# Autodesk Inventor assembly: linear-guide-Hand
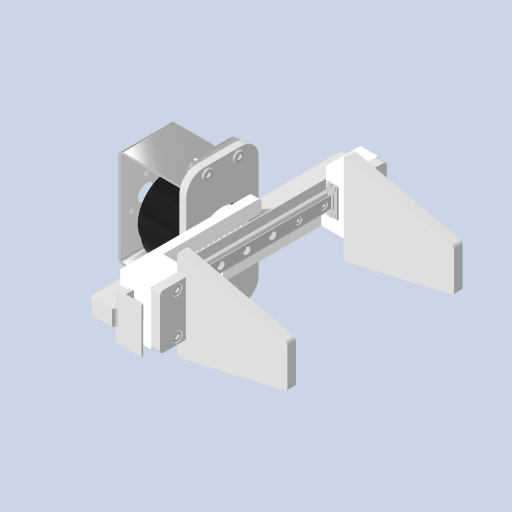
[picture p0: Inventor's stored thumbnail of the model, 512x512]
Saved by Autodesk Inventor 2023 (Build 270158000, 158)
## iProperties
Category: PARTsolutions
Company: MISUMI
Created: 2024-12-13
Part Number: linear-guide-Hand
Catalog Web Link: www.cadenas.de
Description: SSEBSLZ, SSEBSLZ-MX, SSE2BSLZ, SSE2BSLZ-MX-Miniature Linear Guides - Short Blocks - Light Preload/Slight Clearance - Standard Grade - Configurable
Vendor: MISUMI
Document SubType Name: Assembly
Designer: psAdmin
Manufacturer: MISUMI
Mass: 7.41683 g
Surface Area: 76.377 cm^2
Volume: 7.41683 cm^3
Density: 1 g/cm^3
PSOL_IDENT_0: {$CADENAS_DATA/23d-libs/misumi/metric/06_linear_guides/sebslz_asmtab.prj},252 {VTYP=3D},{STYP=ASSTAB
PSOL_IDENT_1: },{NB=SSE2BSLZ8-140},{LINA=SSE2BSLZ8-140},{NN=SSEBSLZ, SSEBSLZ-MX, SSE2BSLZ, SSE2BSLZ-MX},{DATE=04.0
PSOL_IDENT_2: 4.2024 07:13:14},{GEOMDATE=06.03.2024 06:19:47},{VERSION=},{LINEID=90},{WBVAR=TS,ST,MAT,MX,NOB,GREAS
PSOL_IDENT_3: E,L,ALT1,ALT4},{WBNUMERIC=L}  {NB=SSE2BSLZ8-140},{LINA=SSE2BSLZ8-140},{KT=DUMMY},{PN=SSE2BSLZ8-140},
PSOL_IDENT_4: {RT=B},{TS=Z},{TS1= 'Z','Standard' },{ST=S},{ST1='S', 'w/o Surface Treatment'},{TYPE=SSE2BSLZ},{MAT=
PSOL_IDENT_5: S},{MX=},{MXALG= '','w/o MX(Lubrication unit)' },{NOB=2},{H=8},{GREASE=},{GREASEALG='','Normal', 'L'
PSOL_IDENT_6: , 'L Type Greased ', 'G', 'G Type Greased', 'Y', 'Y Type Greased', 'H', 'H Type Greased'},{LT=Confi
PSOL_IDENT_7: gurable},{L=140},{HARD=56HRC~},{W=17},{L1=19.6},{B=12},{C=8},{SLL=M2x2.5},{L2=9.6},{K=6.5},{CBB=0.3}
PSOL_IDENT_8: ,{W1=7},{W2=5.0},{H1=4.7},{CAA=0.3},{DD1DD2HH=2.4x4.2x2.3},{F=15},{G=10},{ALT1=},{ALT1ALG= '', 'w/o
PSOL_IDENT_9: MC (Tapped Holes)' },{MC=M3},{MC1=3.0},{M=9},{LL=L},{L0=[56:69/1],[71:84/1],[86:99/1],[101:114/1],[1
PSOL_IDENT_10: 16:129/1],[131:144/1],[146:159/1],[161:174/1],[176:189/1],[191:204/1],[206:219/1],[221:234/1],[236:2
PSOL_IDENT_11: 49/1],[251:264/1],[266:279/1],[281:294/1],[296:309/1]},{REC1=   '','N/A'    },{ALT4=},{ALT4ALG= '','
PSOL_IDENT_12: N/A' },{PPATH=sebslz_series/sebslz_asmtpl.prj}
NB: SSE2BSLZ8-140
NN: SSEBSLZ, SSEBSLZ-MX, SSE2BSLZ, SSE2BSLZ-MX
NT: Miniature Linear Guides - Short Blocks - Light Preload/Slight Clearance - Standard Grade - Configurable
NBSYN: $PN.
LINA: SSE2BSLZ8-140
CATALOG: Misumi
PN: SSE2BSLZ8-140
MAT: Stainless Steel
MX: w/o MX(Lubrication unit)
NOB: 2
H: 8
GREASE: Normal
L: 140
W: 17
L1: 19.6
B: 12
C: 8
SLL: M2x2.5
L2: 9.6
K: 6.5
CBB: 0.3
W1: 7
W2: 5
H1: 4.7
CAA: 0.3
DD1DD2HH: 2.4x4.2x2.3
F: 15
G: 10
ALT1: w/o MC (Tapped Holes)
ALT4: N/A
SUPPLIER: MISUMI
ARTICLENO: SSE2BSLZ8-140
BOMINFO: SSE2BSLZ8-140
CREATOR: CADENAS GmbH
Title: SSE2BSLZ8-140
Author: Cadenas PARTsolutions
Comments: Miniature Linear Guides - Short Blocks - Light Preload/Slight Clearance - Standard Grade - Configurable
## Documents named in this file (16)
- D:\GitHub\inventor\syu-si\OfficeRobot\Hand\linear-guide-Hand.iam
- D:\GitHub\inventor\syu-si\OfficeRobot\ReadyMade\linear_guide\SSE2BSLZ8-140\SSE2BLZ8-140_r1.ipt
- D:\GitHub\inventor\syu-si\OfficeRobot\ReadyMade\linear_guide\SSE2BSLZ8-140\SEBSZ8_b.ipt
- D:\GitHub\inventor\syu-si\OfficeRobot\ReadyMade\linear_guide\SSE2BSLZ8-140\BOLT2-6.ipt
- D:\GitHub\inventor\syu-si\OfficeRobot\Hand\linear-gear.ipt
- D:\GitHub\inventor\syu-si\OfficeRobot\ReadyMade\Screw\CSH-316L-M2-6.ipt
- D:\GitHub\inventor\syu-si\OfficeRobot\Hand\fix-guide-motor.ipt
- D:\GitHub\inventor\syu-si\OfficeRobot\Hand\hand-gear.ipt
- D:\GitHub\inventor\syu-si\OfficeRobot\ReadyMade\Steadywin\GIM3505-8_with-driver.ipt
- D:\GitHub\inventor\syu-si\OfficeRobot\ReadyMade\Screw\CSH-316L-M2_5-6.ipt
- D:\GitHub\inventor\syu-si\OfficeRobot\Hand\sheet.ipt
- D:\GitHub\inventor\syu-si\OfficeRobot\Hand\hand_box2.ipt
- D:\GitHub\inventor\syu-si\OfficeRobot\Hand\nail.ipt
- D:\GitHub\inventor\syu-si\OfficeRobot\ReadyMade\Screw\FB-305530.ipt
- D:\GitHub\inventor\syu-si\OfficeRobot\ReadyMade\Screw\CBE3-5.ipt
- D:\GitHub\inventor\syu-si\OfficeRobot\ReadyMade\Screw\FB-2001.ipt
## Components (43 placed, 15 different names)
1. SSE2BLZ8-140_r1:1 — to_block_Z@1 <-> to_rail_Z@2, to_block_YZ@1 <-> to_rail_YZ@2, to_block_2_Z@1 <-> to_rail_Z@3, to_block_2_YZ@1 <-> to_rail_YZ@3, to_bolt_1_Z@1 <-> to_cp_Z@4, to_bolt_1_YZ@1 <-> to_cp_YZ@4, to_bolt_2_Z@1 <-> to_cp_Z@5, to_bolt_2_YZ@1 <-> to_cp_YZ@5, to_bolt_3_Z@1 <-> to_cp_Z@6, to_bolt_3_YZ@1 <-> to_cp_YZ@6, to_bolt_7_Z@1 <-> to_cp_Z@10, to_bolt_7_YZ@1 <-> to_cp_YZ@10, to_bolt_8_Z@1 <-> to_cp_Z@11, to_bolt_8_YZ@1 <-> to_cp_YZ@11, to_bolt_9_Z@1 <-> to_cp_Z@12, to_bolt_9_YZ@1 <-> to_cp_YZ@12, 挿入:6, 挿入:7, 挿入:13, 挿入:14, 挿入:15, 挿入:16, 挿入:17, 挿入:18, 挿入:19, 挿入:20
2. SEBSZ8_b:1 — to_block_Z@1 <-> to_rail_Z@2, to_block_YZ@1 <-> to_rail_YZ@2, メイト:15, メイト:16, メイト:17
3. SEBSZ8_b:2 — to_block_2_Z@1 <-> to_rail_Z@3, to_block_2_YZ@1 <-> to_rail_YZ@3, メイト:12, メイト:13, メイト:14
4. BOLT2-6:1 — to_bolt_1_Z@1 <-> to_cp_Z@4, to_bolt_1_YZ@1 <-> to_cp_YZ@4, 挿入:15
5. BOLT2-6:2 — to_bolt_2_Z@1 <-> to_cp_Z@5, to_bolt_2_YZ@1 <-> to_cp_YZ@5, 挿入:16
6. BOLT2-6:3 — to_bolt_3_Z@1 <-> to_cp_Z@6, to_bolt_3_YZ@1 <-> to_cp_YZ@6, 挿入:17
7. BOLT2-6:7 — to_bolt_7_Z@1 <-> to_cp_Z@10, to_bolt_7_YZ@1 <-> to_cp_YZ@10, 挿入:18
8. BOLT2-6:8 — to_bolt_8_Z@1 <-> to_cp_Z@11, to_bolt_8_YZ@1 <-> to_cp_YZ@11, 挿入:19
9. BOLT2-6:9 — to_bolt_9_Z@1 <-> to_cp_Z@12, to_bolt_9_YZ@1 <-> to_cp_YZ@12, 挿入:20
10. linear-gear:1 — メイト:12, メイト:13, メイト:14, 挿入:29, 挿入:30
11. linear-gear:2 — メイト:15, メイト:16, メイト:17, 挿入:27, 挿入:28
12. CSH-316L-M2-6:1
13. CSH-316L-M2-6:2
14. CSH-316L-M2-6:3
15. CSH-316L-M2-6:4
16. fix-guide-motor:1 — 挿入:6, 挿入:7, 挿入:8, 挿入:9, 挿入:10, 挿入:11, 挿入:12, 挿入:21, 挿入:22, 挿入:35, 挿入:36, 挿入:37, 挿入:38, 挿入:43, 挿入:44, 挿入:45, 挿入:46, 挿入:47, 挿入:48
17. 平歯車1:1 — 挿入:5
18. GIM3505-8_with-driver:1 — 挿入:5, 挿入:8, 挿入:9
19. CSH-316L-M2_5-6:1 — 挿入:10
20. CSH-316L-M2_5-6:2 — 挿入:12
21. CSH-316L-M2_5-6:3 — 挿入:11
22. sheet:1 — 挿入:13, 挿入:14
23. hand_box2:1 — 挿入:21, 挿入:22
24. nail:1 — 挿入:33, 挿入:34, 挿入:39, 挿入:40
25. nail:2 — 挿入:31, 挿入:32, 挿入:41, 挿入:42
26. FB-305530:2 — 挿入:30, 挿入:31
27. FB-305530:4 — 挿入:29, 挿入:32
28. FB-305530:5 — 挿入:28, 挿入:34
29. FB-305530:7 — 挿入:27, 挿入:33
30. CBE3-5:1 — 挿入:36
31. CBE3-5:2 — 挿入:35
32. CBE3-5:3 — 挿入:37
33. CBE3-5:4 — 挿入:38
34. CBE3-5:5 — 挿入:39
35. CBE3-5:6 — 挿入:40
36. CBE3-5:7 — 挿入:41
37. CBE3-5:8 — 挿入:42
38. FB-2001:1 — 挿入:48
39. FB-2001:2 — 挿入:47
40. FB-2001:3 — 挿入:46
41. FB-2001:4 — 挿入:45
42. FB-2001:5 — 挿入:44
43. FB-2001:6 — 挿入:43
## Relationships (66: Insert 44, Mate 14, Angle 8)
- to_block_Z@1 <-> to_rail_Z@2 [Mate]: SSE2BLZ8-140_r1:1 ↔ SEBSZ8_b:1
- to_block_YZ@1 <-> to_rail_YZ@2 [Angle] (180 deg): SSE2BLZ8-140_r1:1 ↔ SEBSZ8_b:1
- to_block_2_Z@1 <-> to_rail_Z@3 [Mate]: SSE2BLZ8-140_r1:1 ↔ SEBSZ8_b:2
- to_block_2_YZ@1 <-> to_rail_YZ@3 [Angle] (180 deg): SSE2BLZ8-140_r1:1 ↔ SEBSZ8_b:2
- to_bolt_1_Z@1 <-> to_cp_Z@4 [Mate]: SSE2BLZ8-140_r1:1 ↔ BOLT2-6:1
- to_bolt_1_YZ@1 <-> to_cp_YZ@4 [Angle] (0 deg): SSE2BLZ8-140_r1:1 ↔ BOLT2-6:1
- to_bolt_2_Z@1 <-> to_cp_Z@5 [Mate]: SSE2BLZ8-140_r1:1 ↔ BOLT2-6:2
- to_bolt_2_YZ@1 <-> to_cp_YZ@5 [Angle] (0 deg): SSE2BLZ8-140_r1:1 ↔ BOLT2-6:2
- to_bolt_3_Z@1 <-> to_cp_Z@6 [Mate]: SSE2BLZ8-140_r1:1 ↔ BOLT2-6:3
- to_bolt_3_YZ@1 <-> to_cp_YZ@6 [Angle] (0 deg): SSE2BLZ8-140_r1:1 ↔ BOLT2-6:3
- to_bolt_7_Z@1 <-> to_cp_Z@10 [Mate]: SSE2BLZ8-140_r1:1 ↔ BOLT2-6:7
- to_bolt_7_YZ@1 <-> to_cp_YZ@10 [Angle] (0 deg): SSE2BLZ8-140_r1:1 ↔ BOLT2-6:7
- to_bolt_8_Z@1 <-> to_cp_Z@11 [Mate]: SSE2BLZ8-140_r1:1 ↔ BOLT2-6:8
- to_bolt_8_YZ@1 <-> to_cp_YZ@11 [Angle] (0 deg): SSE2BLZ8-140_r1:1 ↔ BOLT2-6:8
- to_bolt_9_Z@1 <-> to_cp_Z@12 [Mate]: SSE2BLZ8-140_r1:1 ↔ BOLT2-6:9
- to_bolt_9_YZ@1 <-> to_cp_YZ@12 [Angle] (0 deg): SSE2BLZ8-140_r1:1 ↔ BOLT2-6:9
- メイト:12 [Mate]: SEBSZ8_b:2 ↔ linear-gear:1
- メイト:13 [Mate] (0.25 mm): SEBSZ8_b:2 ↔ linear-gear:1
- メイト:14 [Mate]: SEBSZ8_b:2 ↔ linear-gear:1
- メイト:15 [Mate]: SEBSZ8_b:1 ↔ linear-gear:2
- メイト:16 [Mate]: SEBSZ8_b:1 ↔ linear-gear:2
- メイト:17 [Mate] (0.25 mm): SEBSZ8_b:1 ↔ linear-gear:2
- [Insert]: linear-gear:2 ↔ CSH-316L-M2-6:3
- [Insert]: linear-gear:2 ↔ CSH-316L-M2-6:4
- [Insert]: linear-gear:1 ↔ CSH-316L-M2-6:1
- [Insert]: linear-gear:1 ↔ CSH-316L-M2-6:2
- 挿入:5 [Insert]: 平歯車1:1 ↔ GIM3505-8_with-driver:1
- 挿入:6 [Insert] (0.5 mm): SSE2BLZ8-140_r1:1 ↔ fix-guide-motor:1
- 挿入:7 [Insert] (0.5 mm): SSE2BLZ8-140_r1:1 ↔ fix-guide-motor:1
- 挿入:8 [Insert]: fix-guide-motor:1 ↔ GIM3505-8_with-driver:1
- 挿入:9 [Insert]: fix-guide-motor:1 ↔ GIM3505-8_with-driver:1
- 挿入:10 [Insert]: fix-guide-motor:1 ↔ CSH-316L-M2_5-6:1
- 挿入:11 [Insert]: fix-guide-motor:1 ↔ CSH-316L-M2_5-6:3
- 挿入:12 [Insert]: fix-guide-motor:1 ↔ CSH-316L-M2_5-6:2
- 挿入:13 [Insert]: SSE2BLZ8-140_r1:1 ↔ sheet:1
- 挿入:14 [Insert]: SSE2BLZ8-140_r1:1 ↔ sheet:1
- 挿入:15 [Insert]: SSE2BLZ8-140_r1:1 ↔ BOLT2-6:1
- 挿入:16 [Insert]: SSE2BLZ8-140_r1:1 ↔ BOLT2-6:2
- 挿入:17 [Insert]: SSE2BLZ8-140_r1:1 ↔ BOLT2-6:3
- 挿入:18 [Insert]: SSE2BLZ8-140_r1:1 ↔ BOLT2-6:7
- 挿入:19 [Insert]: SSE2BLZ8-140_r1:1 ↔ BOLT2-6:8
- 挿入:20 [Insert]: SSE2BLZ8-140_r1:1 ↔ BOLT2-6:9
- 挿入:21 [Insert]: fix-guide-motor:1 ↔ hand_box2:1
- 挿入:22 [Insert]: fix-guide-motor:1 ↔ hand_box2:1
- 挿入:27 [Insert]: linear-gear:2 ↔ FB-305530:7
- 挿入:28 [Insert]: linear-gear:2 ↔ FB-305530:5
- 挿入:29 [Insert]: linear-gear:1 ↔ FB-305530:4
- 挿入:30 [Insert]: linear-gear:1 ↔ FB-305530:2
- 挿入:31 [Insert]: nail:2 ↔ FB-305530:2
- 挿入:32 [Insert]: nail:2 ↔ FB-305530:4
- 挿入:33 [Insert]: nail:1 ↔ FB-305530:7
- 挿入:34 [Insert]: nail:1 ↔ FB-305530:5
- 挿入:35 [Insert]: fix-guide-motor:1 ↔ CBE3-5:2
- 挿入:36 [Insert]: fix-guide-motor:1 ↔ CBE3-5:1
- 挿入:37 [Insert]: fix-guide-motor:1 ↔ CBE3-5:3
- 挿入:38 [Insert]: fix-guide-motor:1 ↔ CBE3-5:4
- 挿入:39 [Insert]: nail:1 ↔ CBE3-5:5
- 挿入:40 [Insert]: nail:1 ↔ CBE3-5:6
- 挿入:41 [Insert]: nail:2 ↔ CBE3-5:7
- 挿入:42 [Insert]: nail:2 ↔ CBE3-5:8
- 挿入:43 [Insert]: fix-guide-motor:1 ↔ FB-2001:6
- 挿入:44 [Insert]: fix-guide-motor:1 ↔ FB-2001:5
- 挿入:45 [Insert]: fix-guide-motor:1 ↔ FB-2001:4
- 挿入:46 [Insert]: fix-guide-motor:1 ↔ FB-2001:3
- 挿入:47 [Insert]: fix-guide-motor:1 ↔ FB-2001:2
- 挿入:48 [Insert]: fix-guide-motor:1 ↔ FB-2001:1
